# Autodesk Inventor assembly: Assembly1
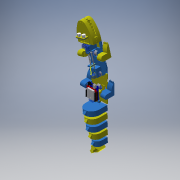
[picture p0: Inventor's stored thumbnail of the model, 180x180]
Saved by Autodesk Inventor 2016 (Build 200138000, 138)
## iProperties
Created: 2017-03-04
Part Number: Assembly1
Document SubType Name: Assembly
Designer: Owner
Author: Owner
## Documents named in this file (34)
- C:\Users\Owner\Documents\Inventor\TSA\2017\Animatronics\Alligator\Alligator\Assembly1.iam
- C:\Users\Owner\Documents\Inventor\TSA\2017\Animatronics\Alligator\Alligator\Frame\Backhalf.ipt
- C:\Users\Owner\Documents\Inventor\TSA\2017\Animatronics\Alligator\Mock Parts\servo (2).ipt
- C:\Users\Owner\Documents\Inventor\TSA\2017\Animatronics\Alligator\Pistons\Syringe1mL\SyringeBody.ipt
- C:\Users\Owner\Documents\Inventor\TSA\2017\Animatronics\Alligator\Alligator\Skin\Skin1.ipt
- C:\Users\Owner\Documents\Inventor\TSA\2017\Animatronics\Alligator\Pistons\Syringe1mL\SyringEnd.ipt
- C:\Users\Owner\Documents\Inventor\TSA\2017\Animatronics\Alligator\Alligator\Tail\Tail1.ipt
- C:\Users\Owner\Documents\Inventor\TSA\2017\Animatronics\Alligator\Alligator\Tail\Tail3.ipt
- C:\Users\Owner\Documents\Inventor\TSA\2017\Animatronics\Alligator\Alligator\Tail\Tail4.ipt
- C:\Users\Owner\Documents\Inventor\TSA\2017\Animatronics\Alligator\Alligator\Tail\Tail5.ipt
- C:\Users\Owner\Documents\Inventor\TSA\2017\Animatronics\Alligator\Alligator\Tail\Tail6.ipt
- C:\Users\Owner\Documents\Inventor\TSA\2017\Animatronics\Alligator\Pistons\PistonTailV2 - Copy\PistonV2.iam
- C:\Users\Owner\Documents\Inventor\TSA\2017\Animatronics\Alligator\Alligator\Reference\Gear.ipt
- C:\Users\Owner\Documents\Inventor\TSA\2017\Animatronics\Alligator\Alligator\Skin\Skin2V2.ipt
- C:\Users\Owner\Documents\Inventor\TSA\2017\Animatronics\Alligator\Alligator\Skin\Skin3.ipt
- C:\Users\Owner\Documents\Inventor\TSA\2017\Animatronics\Alligator\Alligator\Skin\Skin4.ipt
- C:\Users\Owner\Documents\Inventor\TSA\2017\Animatronics\Alligator\Alligator\Frame\LargeConnectorBodies.ipt
- C:\Users\Owner\Documents\Inventor\TSA\2017\Animatronics\Alligator\Alligator\Legs\Leg.ipt
- C:\Users\Owner\Documents\Inventor\D3D Crawl\Movement\Idler Bearing.ipt
- C:\Users\Owner\Documents\Inventor\TSA\2017\Animatronics\Alligator\Alligator\Legs\Leg_MIR.ipt
- C:\Users\Owner\Documents\Inventor\TSA\2017\Animatronics\Alligator\Alligator\Frame\HeadSKin.ipt
- C:\Users\Owner\Documents\Inventor\TSA\2017\Animatronics\Alligator\Alligator\Hinge.ipt
- C:\Users\Owner\Documents\Inventor\TSA\2017\Animatronics\Alligator\Alligator\Toungue.ipt
- C:\Users\Owner\Documents\Inventor\TSA\2017\Animatronics\Alligator\Alligator\Wheel.ipt
- C:\Users\Owner\Documents\Inventor\TSA\2017\Animatronics\Alligator\Mock Parts\HC-SR04.ipt
- C:\Users\Owner\Documents\Inventor\TSA\2017\Animatronics\Alligator\Rack and Pionion\Assembly1.iam
- C:\Users\Owner\Documents\Inventor\TSA\2017\Animatronics\Alligator\Alligator\Frame\HeadFrame.ipt
- C:\Users\Owner\Documents\Inventor\TSA\2017\Animatronics\Alligator\Rack and Pionion\Guide.ipt
- C:\Users\Owner\Documents\Inventor\TSA\2017\Animatronics\Alligator\Alligator\Frame\StupidPiece.ipt
- C:\Users\Owner\Documents\Inventor\TSA\2017\Animatronics\Alligator\Alligator\Frame\Fronthalf1.ipt
- C:\Users\Owner\Documents\Inventor\TSA\2017\Animatronics\Alligator\Alligator\Frame\Fronthalf2.ipt
- C:\Users\Owner\Documents\Inventor\TSA\2017\Animatronics\Alligator\Alligator\Lid.ipt
- C:\Users\Owner\Documents\Inventor\TSA\2017\Animatronics\Alligator\Alligator\Tail\Tail2.ipt
- C:\Users\Owner\Documents\Inventor\TSA\2017\Animatronics\Alligator\Mock Parts\ElectricCore.iam
## Components (48 placed, 33 different names)
1. PistonV2:1 [sub-assembly] — Mate:110, Mate:111, Mate:160, Mate:161, Mate:197
2. Gear:1 — Mate:41, Mate:42
3. servo (2):7 — Mate:41, Mate:42, Flush:120, Flush:121, Mate:154
4. servo (2):8 — Flush:84, Mate:128, Mate:129, Mate:130
5. Toungue:1
6. Wheel:1 — Flush:84
7. HC-SR04:1 — Mate:177, Mate:178, Mate:179
8. Assembly1:1 [sub-assembly] — Mate:110, Mate:111, Mate:117, Tangent:1, Tangent:2, Flush:123, Mate:163
9. SyringeBody:2 — Mate:116
10. SyringEnd:3 — Mate:116, Mate:117, Tangent:1, Tangent:2
11. servo (2):9 — Flush:100, Flush:101, Mate:131, Mate:196
12. Tail3:2 — Mate:191, Mate:192
13. Tail4:2
14. Tail5:2
15. Tail6:2
16. Backhalf:2 — Flush:99, Mate:124, Mate:125, Mate:128, Mate:129, Mate:130, Flush:100, Flush:101, Mate:131, Mate:132, Mate:133, Mate:134, Mate:137, Flush:106, Mate:139, Flush:107, Mate:195
17. StupidPiece:1 — Flush:99, Mate:124, Mate:125, Mate:187, Mate:188
18. LargeConnectorBodies:2 — Mate:132, Mate:133, Mate:134, Mate:136
19. Fronthalf1:1 — Flush:102, Mate:135, Flush:103, Flush:114, Mate:147, Flush:115, Mate:155, Mate:157, Mate:158, Mate:160, Mate:161, Mate:162, Mate:165, Flush:124, Mate:166, Mate:174, Flush:127, Mate:175, Mate:197
20. Fronthalf2:1 — Flush:102, Mate:135, Flush:103, Mate:136, Mate:137, Flush:120, Flush:121, Mate:154
21. Skin4:2 — Flush:104, Flush:105, Mate:138, Flush:107, Flush:108, Flush:110, Flush:111, Mate:145
22. Skin3:2 — Flush:104, Flush:105, Mate:138, Flush:106, Mate:139, Flush:109, Mate:144
23. Skin2V2:2 — Flush:112, Flush:113, Mate:146, Mate:152, Flush:118, Mate:153
24. Skin1:2 — Flush:112, Flush:113, Mate:146, Flush:114, Mate:147, Flush:115, Flush:116, Flush:117, Flush:119
25. Idler Bearing:7
26. Leg:3 — Flush:108, Flush:109, Mate:144
27. Idler Bearing:8 — Mate:194
28. Leg_MIR:3 — Flush:110, Flush:111, Mate:145, Mate:194
29. Idler Bearing:9
30. Leg:4 — Flush:116, Flush:117, Mate:152
31. Idler Bearing:10 — Mate:193
32. Leg_MIR:4 — Flush:118, Mate:153, Flush:119, Mate:193
33. servo (2):10 — Mate:155, Mate:156, Mate:157, Mate:158
34. Wheel:2 — Mate:156
35. Guide:2 — Mate:162, Flush:123, Mate:163
36. SyringeBody:3 — Mate:165, Flush:124, Mate:166
37. SyringEnd:4
38. HeadFrame:2 — Mate:174, Flush:127, Mate:175, Mate:182, Mate:183, Mate:184
39. HeadSKin:2 — Mate:169, Flush:126, Mate:170, Mate:171
40. Lid:1 — Mate:169, Flush:126, Mate:170, Mate:171, Mate:177, Mate:178, Mate:179, Mate:185, Mate:186
41. Toungue:2
42. Toungue:3
43. Toungue:4
44. Toungue:5
45. Hinge:3 — Mate:182, Mate:183, Mate:184, Mate:185, Mate:186
46. Tail1:1 — Mate:187, Mate:188, Mate:189, Mate:190
47. Tail2:1 — Mate:189, Mate:190, Mate:191, Mate:192
48. ElectricCore:1 [sub-assembly] — Mate:195, Mate:196
## Relationships (108: Mate 74, Flush 32, Tangent 2)
- Mate:41: Gear:1 ↔ servo (2):7
- Mate:42: Gear:1 ↔ servo (2):7
- Flush:84: servo (2):8 ↔ Wheel:1
- Mate:110: PistonV2:1 ↔ Assembly1:1
- Mate:111: PistonV2:1 ↔ Assembly1:1
- [Mate]: SyringeBody:2 ↔ SyringEnd:3
- Mate:116: SyringeBody:2 ↔ SyringEnd:3
- Mate:117: Assembly1:1 ↔ SyringEnd:3
- Tangent:1: Assembly1:1 ↔ SyringEnd:3
- Tangent:2: Assembly1:1 ↔ SyringEnd:3
- [Flush]: Tail3:2 ↔ Tail4:2
- [Flush]: Tail4:2 ↔ Tail5:2
- [Flush]: Tail5:2 ↔ Tail6:2
- [Mate]: Tail5:2 ↔ Tail6:2
- [Mate]: Tail4:2 ↔ Tail5:2
- [Mate]: Tail3:2 ↔ Tail4:2
- Flush:99: Backhalf:2 ↔ StupidPiece:1
- Mate:124: Backhalf:2 ↔ StupidPiece:1
- Mate:125 (0.25 mm): Backhalf:2 ↔ StupidPiece:1
- Mate:128: servo (2):8 ↔ Backhalf:2
- Mate:129: servo (2):8 ↔ Backhalf:2
- Mate:130: servo (2):8 ↔ Backhalf:2
- Flush:100: servo (2):9 ↔ Backhalf:2
- Flush:101: servo (2):9 ↔ Backhalf:2
- Mate:131 (0.5 mm): servo (2):9 ↔ Backhalf:2
- Mate:132: Backhalf:2 ↔ LargeConnectorBodies:2
- Mate:133: Backhalf:2 ↔ LargeConnectorBodies:2
- Mate:134: Backhalf:2 ↔ LargeConnectorBodies:2
- Flush:102: Fronthalf1:1 ↔ Fronthalf2:1
- Mate:135: Fronthalf1:1 ↔ Fronthalf2:1
- Flush:103: Fronthalf1:1 ↔ Fronthalf2:1
- Mate:136: LargeConnectorBodies:2 ↔ Fronthalf2:1
- Mate:137: Backhalf:2 ↔ Fronthalf2:1
- Flush:104: Skin4:2 ↔ Skin3:2
- Flush:105: Skin4:2 ↔ Skin3:2
- Mate:138: Skin4:2 ↔ Skin3:2
- Flush:106: Backhalf:2 ↔ Skin3:2
- Mate:139: Backhalf:2 ↔ Skin3:2
- Flush:107: Backhalf:2 ↔ Skin4:2
- [Mate]: Idler Bearing:7 ↔ Leg:3
- [Mate] (0.5 mm): Idler Bearing:7 ↔ Leg:3
- [Mate]: Idler Bearing:8 ↔ Leg_MIR:3
- [Mate] (0.5 mm): Idler Bearing:8 ↔ Leg_MIR:3
- Flush:108: Skin4:2 ↔ Leg:3
- Flush:109: Skin3:2 ↔ Leg:3
- Mate:144 (0.25 mm): Skin3:2 ↔ Leg:3
- Flush:110: Skin4:2 ↔ Leg_MIR:3
- Flush:111: Skin4:2 ↔ Leg_MIR:3
- Mate:145 (0.25 mm): Skin4:2 ↔ Leg_MIR:3
- Flush:112: Skin2V2:2 ↔ Skin1:2
- Flush:113: Skin2V2:2 ↔ Skin1:2
- Mate:146: Skin2V2:2 ↔ Skin1:2
- Flush:114: Fronthalf1:1 ↔ Skin1:2
- Mate:147: Fronthalf1:1 ↔ Skin1:2
- Flush:115: Fronthalf1:1 ↔ Skin1:2
- [Mate]: Idler Bearing:9 ↔ Leg:4
- [Mate] (0.5 mm): Idler Bearing:9 ↔ Leg:4
- [Mate]: Idler Bearing:10 ↔ Leg_MIR:4
- [Mate] (0.5 mm): Idler Bearing:10 ↔ Leg_MIR:4
- Flush:116: Skin1:2 ↔ Leg:4
- Flush:117: Skin1:2 ↔ Leg:4
- Mate:152 (0.25 mm): Skin2V2:2 ↔ Leg:4
- Flush:118: Skin2V2:2 ↔ Leg_MIR:4
- Mate:153 (0.25 mm): Skin2V2:2 ↔ Leg_MIR:4
- Flush:119: Skin1:2 ↔ Leg_MIR:4
- Flush:120: servo (2):7 ↔ Fronthalf2:1
- Flush:121: servo (2):7 ↔ Fronthalf2:1
- Mate:154 (0.5 mm): servo (2):7 ↔ Fronthalf2:1
- [Flush]: servo (2):10 ↔ Wheel:2
- Mate:155: Fronthalf1:1 ↔ servo (2):10
- Mate:156: servo (2):10 ↔ Wheel:2
- Mate:157: Fronthalf1:1 ↔ servo (2):10
- Mate:158: Fronthalf1:1 ↔ servo (2):10
- Mate:160: PistonV2:1 ↔ Fronthalf1:1
- Mate:161: PistonV2:1 ↔ Fronthalf1:1
- Mate:162: Fronthalf1:1 ↔ Guide:2
- Flush:123: Assembly1:1 ↔ Guide:2
- Mate:163 (0.5 mm): Assembly1:1 ↔ Guide:2
- [Mate]: SyringeBody:3 ↔ SyringEnd:4
- Mate:165: Fronthalf1:1 ↔ SyringeBody:3
- Flush:124: Fronthalf1:1 ↔ SyringeBody:3
- Mate:166: Fronthalf1:1 ↔ SyringeBody:3
- Mate:169: HeadSKin:2 ↔ Lid:1
- Flush:126: HeadSKin:2 ↔ Lid:1
- Mate:170: HeadSKin:2 ↔ Lid:1
- Mate:171 (12.4325 mm): HeadSKin:2 ↔ Lid:1
- Mate:174: Fronthalf1:1 ↔ HeadFrame:2
- Flush:127: Fronthalf1:1 ↔ HeadFrame:2
- Mate:175: Fronthalf1:1 ↔ HeadFrame:2
- Mate:177: HC-SR04:1 ↔ Lid:1
- Mate:178: HC-SR04:1 ↔ Lid:1
- Mate:179: HC-SR04:1 ↔ Lid:1
- Mate:182: HeadFrame:2 ↔ Hinge:3
- Mate:183: HeadFrame:2 ↔ Hinge:3
- Mate:184 (22.6885 mm): HeadFrame:2 ↔ Hinge:3
- Mate:185: Lid:1 ↔ Hinge:3
- Mate:186: Lid:1 ↔ Hinge:3
- Mate:187: StupidPiece:1 ↔ Tail1:1
- Mate:188: StupidPiece:1 ↔ Tail1:1
- Mate:189: Tail1:1 ↔ Tail2:1
- Mate:190: Tail1:1 ↔ Tail2:1
- Mate:191: Tail3:2 ↔ Tail2:1
- Mate:192: Tail3:2 ↔ Tail2:1
- Mate:193: Idler Bearing:10 ↔ Leg_MIR:4
- Mate:194: Idler Bearing:8 ↔ Leg_MIR:3
- Mate:195: Backhalf:2 ↔ ElectricCore:1
- Mate:196: servo (2):9 ↔ ElectricCore:1
- Mate:197: PistonV2:1 ↔ Fronthalf1:1
## Named parameters: d415_d410 = 0 mm, d429_d263 = 0 mm, d430_d264 = 0 mm, d431_d265 = 0 mm, d432_d266 = 0 mm, d433_d267 = 0 mm, d434_d268 = 0 mm, d463_d351 = 0 mm, d464_d354 = 0.5 mm, d465_d352 = 0 mm, d466_d353 = 0.5 mm, d479_d463_d351 = 0 mm, d480_d464_d354 = 0.5 mm, d481_d465_d352 = 0 mm, d482_d466_d353 = 0.5 mm, d492_d394 = 0 mm, d503_d410 = 0 mm
